# Autodesk Inventor assembly: robot
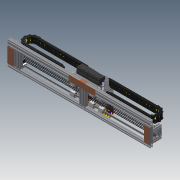
[picture p0: Inventor's stored thumbnail of the model, 180x180]
Saved by Autodesk Inventor 2017 (Build 210142000, 142)
## iProperties
Created: 2018-06-18
Part Number: robot
Document SubType Name: Assembly
Designer: Luiz Gustavo
_SolveAssemblyDoc: Frame Generator Solve Assembly
_Version: 15.0.0
Author: Luiz Gustavo
## Documents named in this file (24)
- C:\Users\Luiz Gustavo\Documents\Inventor\piano-robot\robot.iam
- C:\Users\Luiz Gustavo\Documents\Inventor\piano-robot\eixo-cromado-16h7.ipt
- C:\Users\Luiz Gustavo\Documents\Inventor\piano-robot\conj-mao.iam
- C:\Users\Luiz Gustavo\Documents\Inventor\piano-robot\grabcad\sk16-16mm-shaft-support-1.snapshot.1\sk16.ipt
- C:\Users\Luiz Gustavo\Documents\Inventor\piano-robot\nema23-wotiom.ipt
- C:\Users\Luiz Gustavo\Documents\Inventor\piano-robot\polia-gt2-40t-design1.ipt
- C:\Users\Luiz Gustavo\Documents\Inventor\piano-robot\nema_support_techmakers.ipt
- C:\Users\Luiz Gustavo\Documents\Inventor\piano-robot\robot-frame-reference.ipt
- C:\Users\Luiz Gustavo\Documents\Inventor\piano-robot\robot\Frame\Frame0001.iam
- C:\Users\Luiz Gustavo\Documents\Inventor\piano-robot\grabcad\kfl08-mancal-flange-oval-o8-1.snapshot.1\KFL08 - Mancal Flange oval Ø8.ipt
- C:\Users\Luiz Gustavo\Documents\Inventor\piano-robot\cable-carrier.iam
- C:\Users\Luiz Gustavo\Documents\Inventor\piano-robot\manifold.iam
- C:\Users\Luiz Gustavo\Documents\Inventor\piano-robot\correia-gt2.ipt
- C:\Users\Luiz Gustavo\Documents\Inventor\piano-robot\contra-eixo.ipt
- C:\Users\Luiz Gustavo\Documents\Inventor\piano-robot\robot\Design Accelerator\Bolted Connection1.iam
- C:\Users\Luiz Gustavo\Documents\Inventor\piano-robot\robot\Design Accelerator\Bolted Connection2.iam
- C:\Users\Luiz Gustavo\Documents\Inventor\piano-robot\gabaritos\gabatarito-rolamento.ipt
- C:\Users\Luiz Gustavo\Documents\Inventor\piano-robot\gabaritos\gabarito-30.ipt
- C:\Users\Luiz Gustavo\Documents\Inventor\piano-robot\gabaritos\gabarito-suporte-motor-lateral.ipt
- C:\Users\Luiz Gustavo\Documents\Inventor\piano-robot\gabaritos\gabarito-contraponto.ipt
- C:\Users\Luiz Gustavo\Documents\Inventor\piano-robot\gabaritos\gabarito-suporte-motor-embaixo.ipt
- C:\Users\Luiz Gustavo\Documents\Inventor\piano-robot\gabarito-bloco-solenoide.ipt
- C:\Users\Luiz Gustavo\Documents\Inventor\piano-robot\gabarito-porta-cabos.ipt
- C:\Users\Luiz Gustavo\Documents\Inventor\piano-robot\gabarito-travessa-60.ipt
## Components (39 placed, 22 different names)
1. eixo-cromado-16h7:1 — Mate:1, Mate:2, Mate:3, Cylindrical:1, Cylindrical:2, Rigid:4, Rigid:5
2. eixo-cromado-16h7:2 — Mate:4, Mate:5, Mate:6, Mate:7, Rigid:1, Rigid:3
3. conj-mao:1 [sub-assembly] — Cylindrical:1, Mate:6, Symmetry:1
4. conj-mao:2 [sub-assembly] — Cylindrical:2, Mate:7, Symmetry:1
5. sk16:1 — Rigid:1, Mate:14
6. sk16:2 — Rigid:5, Flush:3, Mate:11, Mate:15
7. sk16:3 — Rigid:4
8. sk16:4 — Rigid:3, Mate:13
9. nema23-wotiom:1 — Rigid:7, Rigid:8, Flush:2
10. nema23-wotiom:2 — Rigid:6, Rigid:9, Flush:2
11. polia-gt2-40t-design1:1 — Rigid:6, Mate:8, Mate:10
12. polia-gt2-40t-design1:2 — Rigid:7, Mate:8, Flush:4
13. polia-gt2-40t-design1:3 — Rigid:10, Mate:20, Mate:22, Mate:31, Mate:32, Rigid:11
14. polia-gt2-40t-design1:4 — Rigid:10, Mate:12, Flush:4, Mate:19, Mate:21, Mate:33, Mate:34, Rigid:12
15. nema_support_techmakers:1 — Rigid:8, Flush:1, Mate:16
16. nema_support_techmakers:2 — Rigid:9, Flush:1, Flush:3, Mate:11, Mate:17, Mate:18
17. robot-frame-reference:1 — Flush:5, Mate:16, Mate:17, Mate:18
18. Frame0001:1 [sub-assembly] — Mate:23, Mate:26, Flush:6, Mate:27, Flush:7, Mate:29, Flush:9, Flush:10, Flush:11, Flush:12, Flush:13, Flush:14, Flush:15, Flush:16, Flush:17
19. cable-carrier:1 [sub-assembly] — Mate:26, Flush:6, Flush:8
20. cable-carrier:2 [sub-assembly] — Mate:27, Flush:7, Mate:28
21. manifold:1 [sub-assembly] — Mate:29, Flush:9, Mate:30
22. correia-gt2:1 — Mate:33, Mate:34
23. correia-gt2:2 — Mate:31, Mate:32
24. KFL08 - Mancal Flange oval Ø8:1 — Mate:19, Mate:21, Mate:23, Mate:24, Mate:25, Symmetry:2, Mate:37, Mate:38, Mate:39
25. KFL08 - Mancal Flange oval Ø8:2 — Mate:20, Mate:22, Mate:24, Mate:25, Symmetry:2, Mate:35, Mate:36, Mate:40
26. KFL08 - Mancal Flange oval Ø8:3 — Mate:37, Mate:38, Mate:39, Mate:45, Mate:46
27. KFL08 - Mancal Flange oval Ø8:4 — Mate:35, Mate:36, Mate:40, Mate:47, Mate:48
28. contra-eixo:1 — Rigid:11
29. contra-eixo:2 — Rigid:12
30. Bolted Connection:1 [sub-assembly] — Mate:45, Mate:46
31. Bolted Connection:2 [sub-assembly] — Mate:47, Mate:48
32. gabatarito-rolamento:1 — Flush:10
33. gabarito-30:1 — Flush:11
34. gabarito-suporte-motor-lateral:1 — Flush:12
35. gabarito-contraponto:1 — Flush:13
36. gabarito-suporte-motor-embaixo:1 — Flush:14
37. gabarito-bloco-solenoide:1 — Flush:15
38. gabarito-porta-cabos:1 — Flush:16
39. gabarito-travessa-60:1 — Flush:17
## Relationships (75: Mate 43, Flush 17, WeldJoint 11, CylindricalJoint 2, Symmetry 2)
- Mate:1: eixo-cromado-16h7:1
- Mate:2: eixo-cromado-16h7:1
- Mate:3: eixo-cromado-16h7:1
- Mate:4: eixo-cromado-16h7:2
- Mate:5: eixo-cromado-16h7:2
- Cylindrical:1: eixo-cromado-16h7:1 ↔ conj-mao:1
- Mate:6: eixo-cromado-16h7:2 ↔ conj-mao:1
- Cylindrical:2: eixo-cromado-16h7:1 ↔ conj-mao:2
- Mate:7: eixo-cromado-16h7:2 ↔ conj-mao:2
- Rigid:1 [WeldJoint]: eixo-cromado-16h7:2 ↔ sk16:1
- Rigid:3 [WeldJoint]: eixo-cromado-16h7:2 ↔ sk16:4
- Rigid:4 [WeldJoint]: eixo-cromado-16h7:1 ↔ sk16:3
- Rigid:5 [WeldJoint]: eixo-cromado-16h7:1 ↔ sk16:2
- Rigid:6 [WeldJoint]: nema23-wotiom:2 ↔ polia-gt2-40t-design1:1
- Rigid:7 [WeldJoint]: nema23-wotiom:1 ↔ polia-gt2-40t-design1:2
- Rigid:8 [WeldJoint]: nema23-wotiom:1 ↔ nema_support_techmakers:1
- Rigid:9 [WeldJoint]: nema23-wotiom:2 ↔ nema_support_techmakers:2
- Mate:8 (2 mm): polia-gt2-40t-design1:1 ↔ polia-gt2-40t-design1:2
- Flush:1: nema_support_techmakers:1 ↔ nema_support_techmakers:2
- Flush:2: nema23-wotiom:1 ↔ nema23-wotiom:2
- Flush:3: sk16:2 ↔ nema_support_techmakers:2
- Symmetry:1: conj-mao:1 ↔ conj-mao:2
- Mate:10 (1 mm): polia-gt2-40t-design1:1
- Mate:11 (1 mm): sk16:2 ↔ nema_support_techmakers:2
- Rigid:10 [WeldJoint] (2 mm): polia-gt2-40t-design1:3 ↔ polia-gt2-40t-design1:4
- Mate:12 (1 mm): polia-gt2-40t-design1:4
- Flush:4: polia-gt2-40t-design1:2 ↔ polia-gt2-40t-design1:4
- Mate:13: sk16:4
- Mate:14: sk16:1
- Mate:15: sk16:2
- Flush:5: robot-frame-reference:1
- Mate:16: nema_support_techmakers:1 ↔ robot-frame-reference:1
- Mate:17: nema_support_techmakers:2 ↔ robot-frame-reference:1
- Mate:18: nema_support_techmakers:2 ↔ robot-frame-reference:1
- Mate:19: polia-gt2-40t-design1:4 ↔ KFL08 - Mancal Flange oval Ø8:1
- Mate:20: polia-gt2-40t-design1:3 ↔ KFL08 - Mancal Flange oval Ø8:2
- Mate:21: polia-gt2-40t-design1:4 ↔ KFL08 - Mancal Flange oval Ø8:1
- Mate:22: polia-gt2-40t-design1:3 ↔ KFL08 - Mancal Flange oval Ø8:2
- Mate:23 (-15 mm): Frame0001:1 ↔ KFL08 - Mancal Flange oval Ø8:1
- Mate:24: KFL08 - Mancal Flange oval Ø8:1 ↔ KFL08 - Mancal Flange oval Ø8:2
- Mate:25 (44 mm): KFL08 - Mancal Flange oval Ø8:1 ↔ KFL08 - Mancal Flange oval Ø8:2
- Symmetry:2: KFL08 - Mancal Flange oval Ø8:1 ↔ KFL08 - Mancal Flange oval Ø8:2
- Mate:26: Frame0001:1 ↔ cable-carrier:1
- Flush:6 (-7 mm): Frame0001:1 ↔ cable-carrier:1
- Mate:27: Frame0001:1 ↔ cable-carrier:2
- Flush:7 (-6.5 mm): Frame0001:1 ↔ cable-carrier:2
- Flush:8 (250 mm): cable-carrier:1
- Mate:28 (250 mm): cable-carrier:2
- Mate:29: Frame0001:1 ↔ manifold:1
- Flush:9: Frame0001:1 ↔ manifold:1
- Mate:30: manifold:1
- Mate:31 (0.5 mm): polia-gt2-40t-design1:3 ↔ correia-gt2:2
- Mate:32: polia-gt2-40t-design1:3 ↔ correia-gt2:2
- Mate:33 (0.5 mm): polia-gt2-40t-design1:4 ↔ correia-gt2:1
- Mate:34: polia-gt2-40t-design1:4 ↔ correia-gt2:1
- Mate:35: KFL08 - Mancal Flange oval Ø8:2 ↔ KFL08 - Mancal Flange oval Ø8:4
- Mate:36: KFL08 - Mancal Flange oval Ø8:2 ↔ KFL08 - Mancal Flange oval Ø8:4
- Mate:37: KFL08 - Mancal Flange oval Ø8:1 ↔ KFL08 - Mancal Flange oval Ø8:3
- Mate:38: KFL08 - Mancal Flange oval Ø8:1 ↔ KFL08 - Mancal Flange oval Ø8:3
- Mate:39 (-36 mm): KFL08 - Mancal Flange oval Ø8:1 ↔ KFL08 - Mancal Flange oval Ø8:3
- Mate:40 (-36 mm): KFL08 - Mancal Flange oval Ø8:2 ↔ KFL08 - Mancal Flange oval Ø8:4
- Rigid:11 [WeldJoint]: polia-gt2-40t-design1:3 ↔ contra-eixo:1
- Rigid:12 [WeldJoint]: polia-gt2-40t-design1:4 ↔ contra-eixo:2
- Mate:45: KFL08 - Mancal Flange oval Ø8:3 ↔ Bolted Connection:1
- Mate:46: KFL08 - Mancal Flange oval Ø8:3 ↔ Bolted Connection:1
- Mate:47: KFL08 - Mancal Flange oval Ø8:4 ↔ Bolted Connection:2
- Mate:48: KFL08 - Mancal Flange oval Ø8:4 ↔ Bolted Connection:2
- Flush:10: Frame0001:1 ↔ gabatarito-rolamento:1
- Flush:11: Frame0001:1 ↔ gabarito-30:1
- Flush:12: Frame0001:1 ↔ gabarito-suporte-motor-lateral:1
- Flush:13: Frame0001:1 ↔ gabarito-contraponto:1
- Flush:14: Frame0001:1 ↔ gabarito-suporte-motor-embaixo:1
- Flush:15: Frame0001:1 ↔ gabarito-bloco-solenoide:1
- Flush:16: Frame0001:1 ↔ gabarito-porta-cabos:1
- Flush:17: Frame0001:1 ↔ gabarito-travessa-60:1
